# Autodesk Inventor assembly: Final Assemblyv2
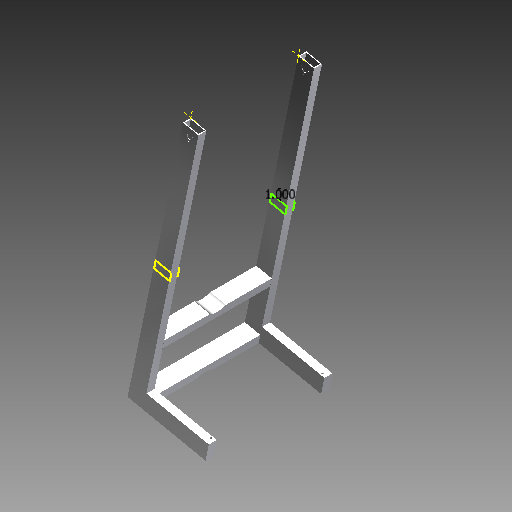
[picture p0: Inventor's stored thumbnail of the model, 512x512]
Saved by Autodesk Inventor 2017 (Build 210142000, 142)
## iProperties
Created: 2018-01-19
Part Number: Final Assemblyv2
Document SubType Name: Assembly
Designer: S331461152
Sending System: Autodesk Inventor 2018
Preprocessor: ST-DEVELOPER v16.13
Title: C:\Users\Steven\Desktop\Good Stuff\Home Stuff\Final Assembly.stp
Author: Steven
## Documents named in this file (4)
- \\ad.ocdsb.ca\studenthome\5\S346795925\Robotics\698590_FRC_Season_2017_18_c6a29b2db01e1b8a_1517863524\Robot Mostly Finalized V16\Final Assemblyv2.iam
- \\ad.ocdsb.ca\studenthome\5\S346795925\Robotics\698590_FRC_Season_2017_18_c6a29b2db01e1b8a_1517863524\Robot Mostly Finalized V16\arm2v2.ipt
- \\ad.ocdsb.ca\studenthome\5\S346795925\Robotics\698590_FRC_Season_2017_18_c6a29b2db01e1b8a_1517863524\Robot Mostly Finalized V16\connectingthing.ipt
- \\ad.ocdsb.ca\studenthome\5\S346795925\Robotics\698590_FRC_Season_2017_18_c6a29b2db01e1b8a_1517863524\Robot Mostly Finalized V16\arm2v2_MIR.ipt
## Components (4 placed, 3 different names)
1. arm2v2:1 — Mate:37, Mate:41
2. connectingthing:1 — Mate:39, Mate:41, Flush:2
3. connectingthing:2 — Mate:37, Flush:1, Mate:42, Flush:2
4. arm2v2_MIR:1 — Mate:39, Flush:1, Mate:42
## Relationships (6: Mate 4, Flush 2)
- Mate:37: arm2v2:1 ↔ connectingthing:2
- Mate:39: connectingthing:1 ↔ arm2v2_MIR:1
- Mate:41: arm2v2:1 ↔ connectingthing:1
- Flush:1: connectingthing:2 ↔ arm2v2_MIR:1
- Mate:42: connectingthing:2 ↔ arm2v2_MIR:1
- Flush:2 (177.8 mm): connectingthing:1 ↔ connectingthing:2
